# Autodesk Inventor assembly: SumoBot
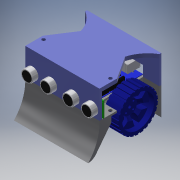
[picture p0: Inventor's stored thumbnail of the model, 180x180]
Saved by Autodesk Inventor 2017 (Build 210142000, 142)
## iProperties
Created: 2018-03-02
Part Number: SumoBot
Document SubType Name: Assembly
Designer: bradl
Author: bradl
## Documents named in this file (15)
- C:\Users\bradl\OneDrive\Documents\McMaster\SUMOBOT\SumoBot.iam
- C:\Users\bradl\OneDrive\Documents\McMaster\SUMOBOT\n20-micro-metal-gearmotor-1.snapshot.2\Inventor\Assembly1\Design Accelerator\Chasis_base.ipt
- C:\Users\bradl\OneDrive\Documents\McMaster\SUMOBOT\n20-micro-metal-gearmotor-1.snapshot.2\Inventor\Mount.ipt
- C:\Users\bradl\OneDrive\Documents\McMaster\SUMOBOT\n20-micro-metal-gearmotor-1.snapshot.2\motor.ipt
- C:\Users\bradl\OneDrive\Documents\McMaster\SUMOBOT\623-zz-bearing-w-o-balls-1.snapshot.5\-bearing mr623zz\-MR623ZZ-assem.iam
- C:\Users\bradl\OneDrive\Documents\McMaster\SUMOBOT\n20-micro-metal-gearmotor-1.snapshot.2\n20_gearbox.ipt
- C:\Users\bradl\OneDrive\Documents\McMaster\SUMOBOT\n20-micro-metal-gearmotor-1.snapshot.2\n20_shaft.ipt
- C:\Users\bradl\OneDrive\Documents\McMaster\SUMOBOT\n20-micro-metal-gearmotor-1.snapshot.2\Inventor\Wheel Mount.ipt
- C:\Users\bradl\OneDrive\Documents\McMaster\SUMOBOT\n20-micro-metal-gearmotor-1.snapshot.2\Inventor\Shaft.ipt
- C:\Users\bradl\OneDrive\Documents\McMaster\SUMOBOT\n20-micro-metal-gearmotor-1.snapshot.2\Inventor\Assembly1\Design Accelerator\Spur Gear16.ipt
- C:\Users\bradl\OneDrive\Documents\McMaster\SUMOBOT\n20-micro-metal-gearmotor-1.snapshot.2\Inventor\Assembly1\Design Accelerator\Spur Gear26.ipt
- C:\Users\bradl\OneDrive\Documents\McMaster\SUMOBOT\n20-micro-metal-gearmotor-1.snapshot.2\Inventor\Wheel2.ipt
- C:\Users\bradl\OneDrive\Documents\McMaster\SUMOBOT\arduino-uno.snapshot.3\arduino uno.iam
- C:\Users\bradl\OneDrive\Documents\McMaster\SUMOBOT\n20-micro-metal-gearmotor-1.snapshot.2\Inventor\Assembly1\Design Accelerator\Chasis_top.ipt
- C:\Users\bradl\OneDrive\Documents\McMaster\SUMOBOT\UltraSonic HC-SR04\Ultra\Ultraconico.ipt
## Components (22 placed, 14 different names)
1. Chasis_base:1 — Flush:1, Mate:1, Mate:2, Mate:3, Mate:4, Mate:5, Mate:6, Mate:7, Mate:8, Mate:9, Flush:4, Flush:5, Mate:10, Angle:1, Angle:2, Mate:11, Flush:6, Flush:14, Mate:39, Flush:15, Flush:16, Flush:17
2. Mount:1 — Mate:1, Mate:3, Mate:4, Flush:3, Tangent:2, Angle:3
3. Mount:2 — Mate:2, Mate:5, Mate:6, Flush:2, Tangent:1, Angle:4
4. motor:1 — Mate:8, Flush:3, Tangent:2, Mate:12, Mate:13
5. motor:2 — Flush:2, Mate:7, Tangent:1, Mate:14, Mate:15
6. -MR623ZZ-assem:1 [sub-assembly] — Mate:9, Flush:4, Angle:1
7. -MR623ZZ-assem:2 [sub-assembly] — Flush:5, Mate:10, Angle:2, Mate:22, Flush:9
8. n20_gearbox:1 — Mate:12, Angle:3, Mate:13, Flush:8, Mate:17
9. n20_gearbox:2 — Mate:14, Angle:4, Mate:15, Flush:13, Mate:33
10. n20_shaft:1 — Flush:13, Mate:33, Mate:34, Angle:12, Mate:35, Mate:36
11. n20_shaft:2 — Flush:8, Mate:17, Mate:25, Angle:10
12. Wheel Mount:1 — Mate:26, Angle:11, Flush:12, Mate:28, Mate:29
13. Shaft:1 — Mate:22, Flush:9, Mate:23, Mate:24, Flush:10, Mate:26, Angle:11, Flush:12, Mate:27
14. Spur Gear1:1 — Mate:23, Mate:24, Flush:10, Flush:11, Rotation:1
15. Spur Gear2:1 — Mate:25, Angle:10, Flush:11, Rotation:1
16. Wheel2:1 — Mate:27, Mate:28, Mate:29
17. Wheel Mount:2 — Mate:34, Angle:12, Mate:35, Mate:37, Mate:38
18. Wheel2:2 — Mate:36, Mate:37, Mate:38
19. arduino uno:1 [sub-assembly] — Flush:14, Mate:39, Flush:15
20. Chasis_top:1 — Flush:16, Flush:17, Mate:41, Mate:42, Flush:18, Mate:43, Mate:44, Flush:19
21. Ultraconico:1 — Mate:41, Mate:42, Flush:18
22. Ultraconico:2 — Mate:43, Mate:44, Flush:19
## Relationships (63: Mate 35, Flush 18, Angle 7, Tangent 2, RelateRotation 1)
- Flush:1: Chasis_base:1
- Mate:1: Chasis_base:1 ↔ Mount:1
- Mate:2: Chasis_base:1 ↔ Mount:2
- Mate:3: Chasis_base:1 ↔ Mount:1
- Mate:4: Chasis_base:1 ↔ Mount:1
- Mate:5: Chasis_base:1 ↔ Mount:2
- Mate:6: Chasis_base:1 ↔ Mount:2
- Flush:2: Mount:2 ↔ motor:2
- Mate:7: Chasis_base:1 ↔ motor:2
- Tangent:1: Mount:2 ↔ motor:2
- Mate:8: Chasis_base:1 ↔ motor:1
- Flush:3: Mount:1 ↔ motor:1
- Tangent:2: Mount:1 ↔ motor:1
- Mate:9: Chasis_base:1 ↔ -MR623ZZ-assem:1
- Flush:4: Chasis_base:1 ↔ -MR623ZZ-assem:1
- Flush:5: Chasis_base:1 ↔ -MR623ZZ-assem:2
- Mate:10: Chasis_base:1 ↔ -MR623ZZ-assem:2
- Angle:1 (0 deg): Chasis_base:1 ↔ -MR623ZZ-assem:1
- Angle:2 (0 deg): Chasis_base:1 ↔ -MR623ZZ-assem:2
- Mate:11: Chasis_base:1
- Flush:6: Chasis_base:1
- Mate:12: motor:1 ↔ n20_gearbox:1
- Angle:3 (0 deg): Mount:1 ↔ n20_gearbox:1
- Mate:13: motor:1 ↔ n20_gearbox:1
- Mate:14: motor:2 ↔ n20_gearbox:2
- Angle:4 (0 deg): Mount:2 ↔ n20_gearbox:2
- Mate:15: motor:2 ↔ n20_gearbox:2
- Flush:8: n20_gearbox:1 ↔ n20_shaft:2
- Mate:17: n20_gearbox:1 ↔ n20_shaft:2
- Mate:22: -MR623ZZ-assem:2 ↔ Shaft:1
- Flush:9: -MR623ZZ-assem:2 ↔ Shaft:1
- Mate:23: Shaft:1 ↔ Spur Gear1:1
- Mate:24: Shaft:1 ↔ Spur Gear1:1
- Flush:10: Shaft:1 ↔ Spur Gear1:1
- Mate:25: n20_shaft:2 ↔ Spur Gear2:1
- Angle:10 (180 deg): n20_shaft:2 ↔ Spur Gear2:1
- Flush:11: Spur Gear1:1 ↔ Spur Gear2:1
- Rotation:1 [RelateRotation] (1 ul): Spur Gear1:1 ↔ Spur Gear2:1
- Mate:26: Wheel Mount:1 ↔ Shaft:1
- Angle:11 (45 deg): Wheel Mount:1 ↔ Shaft:1
- Flush:12: Wheel Mount:1 ↔ Shaft:1
- Mate:27: Shaft:1 ↔ Wheel2:1
- Mate:28: Wheel Mount:1 ↔ Wheel2:1
- Mate:29: Wheel Mount:1 ↔ Wheel2:1
- Flush:13: n20_gearbox:2 ↔ n20_shaft:1
- Mate:33: n20_gearbox:2 ↔ n20_shaft:1
- Mate:34: n20_shaft:1 ↔ Wheel Mount:2
- Angle:12 (45 deg): n20_shaft:1 ↔ Wheel Mount:2
- Mate:35: n20_shaft:1 ↔ Wheel Mount:2
- Mate:36: n20_shaft:1 ↔ Wheel2:2
- Mate:37: Wheel Mount:2 ↔ Wheel2:2
- Mate:38: Wheel Mount:2 ↔ Wheel2:2
- Flush:14: Chasis_base:1 ↔ arduino uno:1
- Mate:39: Chasis_base:1 ↔ arduino uno:1
- Flush:15: Chasis_base:1 ↔ arduino uno:1
- Flush:16: Chasis_base:1 ↔ Chasis_top:1
- Flush:17: Chasis_base:1 ↔ Chasis_top:1
- Mate:41: Chasis_top:1 ↔ Ultraconico:1
- Mate:42: Chasis_top:1 ↔ Ultraconico:1
- Flush:18 (-7.62 mm): Chasis_top:1 ↔ Ultraconico:1
- Mate:43: Chasis_top:1 ↔ Ultraconico:2
- Mate:44: Chasis_top:1 ↔ Ultraconico:2
- Flush:19 (-7.62 mm): Chasis_top:1 ↔ Ultraconico:2
